# Autodesk Inventor assembly: Relaismodul
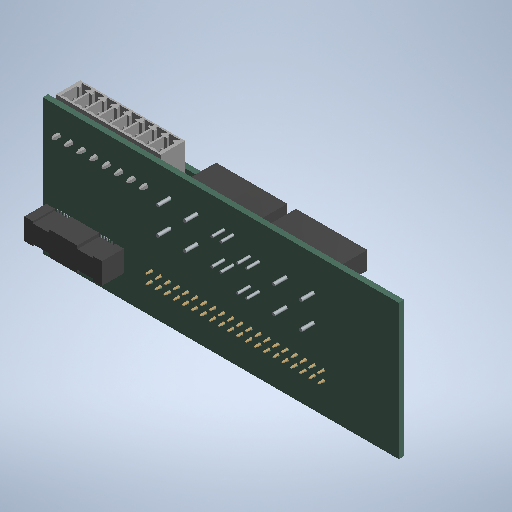
[picture p0: Inventor's stored thumbnail of the model, 512x512]
Saved by Autodesk Inventor 2025.2 (Build 292293000, 293)
## iProperties
Company: Kicad
Created: 2025-07-30
Part Number: Relaismodul
Description: KiCad electronic assembly
Document SubType Name: Baugruppe
Designer: leowa
Authority: Unknown
Title: Relaismodul.step
Author: Pcbnew
Sending System: KiCad to STEP converter
Preprocessor: Open CASCADE STEP processor 7.8
## Documents named in this file (10)
- C:\Users\leowa\OneDrive - Fachhochschule Aachen\FH\8. Semester\CAN Tram CAD\Platinen\Relaismodul\Relaismodul\Relaismodul.iam
- C:\Users\leowa\OneDrive - Fachhochschule Aachen\FH\8. Semester\CAN Tram CAD\Platinen\Relaismodul\Relaismodul\658855603040.iam
- C:\Users\leowa\OneDrive - Fachhochschule Aachen\FH\8. Semester\CAN Tram CAD\Platinen\Relaismodul\Relaismodul\R_1206_3216Metric.ipt
- C:\Users\leowa\OneDrive - Fachhochschule Aachen\FH\8. Semester\CAN Tram CAD\Platinen\Relaismodul\Relaismodul\39502-1008.iam
- C:\Users\leowa\OneDrive - Fachhochschule Aachen\FH\8. Semester\CAN Tram CAD\Platinen\Relaismodul\Relaismodul\PinSocket_2x20_P2.54mm_Vertical.ipt
- C:\Users\leowa\OneDrive - Fachhochschule Aachen\FH\8. Semester\CAN Tram CAD\Platinen\Relaismodul\Relaismodul\156120GS75000.iam
- C:\Users\leowa\OneDrive - Fachhochschule Aachen\FH\8. Semester\CAN Tram CAD\Platinen\Relaismodul\Relaismodul\PCN-105D3MHZ.iam
- C:\Users\leowa\OneDrive - Fachhochschule Aachen\FH\8. Semester\CAN Tram CAD\Platinen\Relaismodul\Relaismodul\2N7002K.iam
- C:\Users\leowa\OneDrive - Fachhochschule Aachen\FH\8. Semester\CAN Tram CAD\Platinen\Relaismodul\Relaismodul\Relaismodul_PCB.ipt
- C:\Users\leowa\OneDrive - Fachhochschule Aachen\FH\8. Semester\CAN Tram CAD\Platinen\Relaismodul Adapter\Relaismodul Adapter\Relaismodul Adapter.iam
## Components (27 placed, 27 different names)
1. 4 [sub-assembly]
2. 5
3. 6
4. 7
5. 8
6. 9
7. 12 [sub-assembly]
8. 13 — Fluchtend:1, Passend:1, Fluchtend:2
9. 16 [sub-assembly]
10. 19 [sub-assembly]
11. 23 [sub-assembly]
12. 24
13. 25 [sub-assembly]
14. 26
15. 27
16. 28 [sub-assembly]
17. 29 [sub-assembly]
18. 30
19. 31 [sub-assembly]
20. 32
21. 33
22. 34
23. 35
24. 36 [sub-assembly]
25. 37 [sub-assembly]
26. 38
27. Relaismodul Adapter:1 [sub-assembly] — Fluchtend:1, Passend:1, Fluchtend:2
## Relationships (3: Flush 2, Mate 1)
- Fluchtend:1 [Flush]: 13 ↔ Relaismodul Adapter:1
- Passend:1 [Mate]: 13 ↔ Relaismodul Adapter:1
- Fluchtend:2 [Flush]: 13 ↔ Relaismodul Adapter:1
